# Autodesk Inventor assembly: oska-assembly
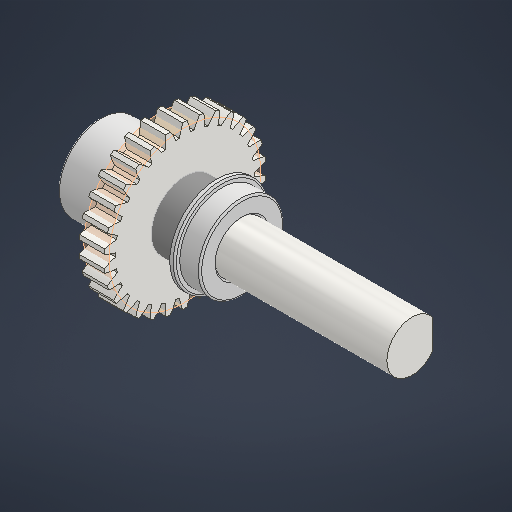
[picture p0: Inventor's stored thumbnail of the model, 512x512]
Saved by Autodesk Inventor 2026.2 (Build 302298000, 298)
## iProperties
Created: 2026-03-09
Part Number: oska-assembly
Document SubType Name: Assembly
Designer: szymo
Author: szymo
## Documents named in this file (7)
- C:\Users\szymo\Downloads\evangelion-turbo\inventor-project\oska-assembly.iam
- C:\Users\szymo\Downloads\evangelion-turbo\inventor-project\shaft.ipt
- C:\Users\szymo\Downloads\evangelion-turbo\inventor-project\BigGear.iam
- C:\Users\szymo\Downloads\evangelion-turbo\inventor-project\ball-bearing.ipt
- C:\Users\szymo\Downloads\evangelion-turbo\inventor-project\flange_bearing.ipt
- C:\Users\szymo\Downloads\evangelion-turbo\inventor-project\radial_magnet.ipt
- C:\Users\szymo\Downloads\evangelion-turbo\inventor-project\steel_spacer.ipt
## Components (6 placed, 6 different names)
1. Shaft:1 — Mate:1, Mate:2, Mate:3, Mate:6, Mate:9
2. Spur Gears:1 [sub-assembly] — Mate:1, Mate:2, Mate:5, Mate:7, Mate:11
3. ball-bearing:2 — Mate:3, Mate:5
4. flange_bearing:1 — Mate:6, Mate:7
5. radial_magnet:1 — Mate:8, Mate:9
6. steel_spacer:1 — Mate:10, Mate:11
## Relationships (10: Mate 10)
- Mate:1: Shaft:1 ↔ Spur Gears:1
- Mate:2: Shaft:1 ↔ Spur Gears:1
- Mate:3: Shaft:1 ↔ ball-bearing:2
- Mate:5 (0.1 mm): Spur Gears:1 ↔ ball-bearing:2
- Mate:6: Shaft:1 ↔ flange_bearing:1
- Mate:7 (3.8 mm): Spur Gears:1 ↔ flange_bearing:1
- Mate:8: radial_magnet:1
- Mate:9 (0.6 mm): Shaft:1 ↔ radial_magnet:1
- Mate:10: steel_spacer:1
- Mate:11: Spur Gears:1 ↔ steel_spacer:1
